# Autodesk Inventor assembly: CuttingHead
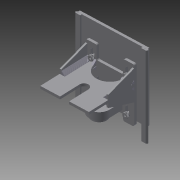
[picture p0: Inventor's stored thumbnail of the model, 180x180]
Saved by Autodesk Inventor 2013 (Build 170138000, 138)
## iProperties
Created: 2012-12-07
Part Number: CuttingHead
Document SubType Name: Assembly
Designer: istvan.burbank
Mass: 179.257 g
Surface Area: 890.164 cm^2
Volume: 179.257 cm^3
Density: 1 g/cm^3
Author: istvan.burbank
## Documents named in this file (8)
- C:\Users\istvan.burbank\Documents\GitHub\Crown-Fire\CAD\CuttingHead\CuttingHead.iam
- C:\Users\istvan.burbank\Documents\GitHub\Crown-Fire\CAD\CuttingHead\AcmeRoundNut.ipt
- C:\Users\istvan.burbank\Documents\GitHub\Crown-Fire\CAD\CuttingHead\AcmeMountingFlange.ipt
- C:\Users\istvan.burbank\Documents\GitHub\Crown-Fire\CAD\CuttingHead\backPlate.ipt
- C:\Users\istvan.burbank\Documents\GitHub\Crown-Fire\CAD\CuttingHead\vee-track.ipt
- D:\GitHub\Crown-Fire\CAD\Templates\vee-track.ipt
- C:\Users\istvan.burbank\Documents\GitHub\Crown-Fire\CAD\Hardware\z-axisSliderShoulderBolts.ipt
- C:\Users\istvan.burbank\Documents\GitHub\Crown-Fire\CAD\CuttingHead\torchArm.iam
## Components (10 placed, 6 different names)
1. AcmeRoundNut:1 — Mate:1, Mate:2
2. AcmeMountingFlange:1 — Mate:1, Mate:2, Mate:3, Flush:3
3. backPlate:1 — Mate:3, Mate:4, Mate:5, Mate:6, Mate:7, Flush:1, Flush:2, Flush:3, Mate:8, Mate:9, Mate:10, Mate:11, Mate:12
4. vee-track:1 — Mate:4, Mate:7, Flush:1
5. vee-track:2 — Mate:5, Mate:6, Flush:2
6. z-axisSliderShoulderBolts:1 — Mate:8, Tangent:1
7. z-axisSliderShoulderBolts:2 — Mate:9, Tangent:3
8. z-axisSliderShoulderBolts:3 — Mate:10, Tangent:2
9. z-axisSliderShoulderBolts:4 — Mate:11, Tangent:4
10. torchArm:1 [sub-assembly] — Tangent:1, Tangent:2, Tangent:3, Tangent:4, Mate:12
## Relationships (19: Mate 12, Tangent 4, Flush 3)
- Mate:1: AcmeRoundNut:1 ↔ AcmeMountingFlange:1
- Mate:2: AcmeRoundNut:1 ↔ AcmeMountingFlange:1
- Mate:3: AcmeMountingFlange:1 ↔ backPlate:1
- Mate:4: backPlate:1 ↔ vee-track:1
- Mate:5: backPlate:1 ↔ vee-track:2
- Mate:6: backPlate:1 ↔ vee-track:2
- Mate:7: backPlate:1 ↔ vee-track:1
- Flush:1: backPlate:1 ↔ vee-track:1
- Flush:2: backPlate:1 ↔ vee-track:2
- Flush:3 (-6.35 mm): AcmeMountingFlange:1 ↔ backPlate:1
- Mate:8: backPlate:1 ↔ z-axisSliderShoulderBolts:1
- Mate:9: backPlate:1 ↔ z-axisSliderShoulderBolts:2
- Mate:10: backPlate:1 ↔ z-axisSliderShoulderBolts:3
- Mate:11: backPlate:1 ↔ z-axisSliderShoulderBolts:4
- Tangent:1: z-axisSliderShoulderBolts:1 ↔ torchArm:1
- Tangent:2: z-axisSliderShoulderBolts:3 ↔ torchArm:1
- Tangent:3: z-axisSliderShoulderBolts:2 ↔ torchArm:1
- Tangent:4: z-axisSliderShoulderBolts:4 ↔ torchArm:1
- Mate:12: backPlate:1 ↔ torchArm:1
